# Autodesk Inventor assembly: Cate2inchMecanum
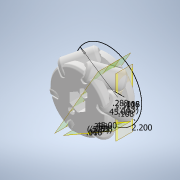
[picture p0: Inventor's stored thumbnail of the model, 180x180]
Saved by Autodesk Inventor 2020 (Build 240168000, 168)
## iProperties
Created: 2020-01-20
Part Number: Cate2inchMecanum
Document SubType Name: Assembly
Designer: srini
Author: srini
## Documents named in this file (3)
- C:\Users\srini\Documents\FRC\2020\IntakeShooter\Cate2inchMecanum.iam
- C:\Users\srini\Documents\FRC\2020\IntakeShooter\Cate2inchMecanumA.ipt
- C:\Users\srini\Documents\FRC\2020\IntakeShooter\Cate2InchMecRoller.ipt
## Components (8 placed, 2 different names)
1. Cate2inchMecanumA:1 — Insert:1, Insert:2, Flush:1
2. Cate2inchMecanumA:2 — Insert:1, Insert:2, Insert:3, Insert:4, Insert:5, Insert:6, Insert:7
3. Cate2InchMecRoller:1 — Flush:1
4. Cate2InchMecRoller:2 — Insert:3
5. Cate2InchMecRoller:3 — Insert:4
6. Cate2InchMecRoller:4 — Insert:5
7. Cate2InchMecRoller:5 — Insert:6
8. Cate2InchMecRoller:6 — Insert:7
## Relationships (8: Insert 7, Flush 1)
- Insert:1: Cate2inchMecanumA:1 ↔ Cate2inchMecanumA:2
- Insert:2: Cate2inchMecanumA:1 ↔ Cate2inchMecanumA:2
- Flush:1: Cate2inchMecanumA:1 ↔ Cate2InchMecRoller:1
- Insert:3 (0.1524 mm): Cate2inchMecanumA:2 ↔ Cate2InchMecRoller:2
- Insert:4 (0.1524 mm): Cate2inchMecanumA:2 ↔ Cate2InchMecRoller:3
- Insert:5 (0.1524 mm): Cate2inchMecanumA:2 ↔ Cate2InchMecRoller:4
- Insert:6 (0.1524 mm): Cate2inchMecanumA:2 ↔ Cate2InchMecRoller:5
- Insert:7 (0.1524 mm): Cate2inchMecanumA:2 ↔ Cate2InchMecRoller:6
